# Autodesk Inventor assembly: A2017_T2_13
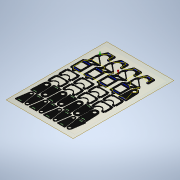
[picture p0: Inventor's stored thumbnail of the model, 180x180]
Saved by Autodesk Inventor 2020 (Build 240168000, 168)
## iProperties
Created: 2021-08-27
Part Number: A2017_T2_13
Document SubType Name: Assembly
Designer: Masato
Author: Masato
## Documents named in this file (6)
- D:\GitHub\inventor\SUSTAINA-OP\Cam\A2017_T2_13.iam
- D:\GitHub\inventor\SUSTAINA-OP\Cam\DisposableBoard.ipt
- D:\GitHub\inventor\SUSTAINA-OP\LowerBody\Foot\Foot_front_frame.ipt
- D:\GitHub\inventor\SUSTAINA-OP\LowerBody\Foot\Foot_back_frame.ipt
- D:\GitHub\inventor\SUSTAINA-OP\LowerBody\Ankle\Ankle_side_frame.ipt
- D:\GitHub\inventor\SUSTAINA-OP\LowerBody\Ankle\Ankle_back_frame.ipt
## Components (29 placed, 5 different names)
1. DisposableBoard:1 — メイト:2, メイト:1, フラッシュ:1, フラッシュ:2, メイト:4, メイト:5, メイト:6, メイト:7, 正接:1, メイト:9, メイト:10, メイト:11, メイト:12, メイト:13, メイト:15, メイト:16, メイト:18, メイト:21
2. Foot_back_frame:7 — メイト:18, メイト:19, メイト:20
3. Foot_back_frame:8 — メイト:21, メイト:22, メイト:23
4. Foot_front_frame:2 — メイト:7, メイト:8, 正接:1, 正接:3
5. Foot_front_frame:1 — メイト:4, メイト:5, メイト:6, メイト:8, 正接:2
6. Foot_front_frame:3
7. Foot_front_frame:4
8. Foot_front_frame:5
9. Foot_front_frame:6
10. Foot_front_frame:7 — メイト:19
11. Foot_front_frame:8
12. Foot_back_frame:1 — メイト:10, メイト:14, 正接:3
13. Foot_back_frame:2 — メイト:9, 正接:2, メイト:13, メイト:14, 正接:4
14. Foot_back_frame:3
15. Foot_back_frame:4
16. Foot_back_frame:5 — メイト:20
17. Foot_back_frame:6
18. Ankle_back_frame:1 — メイト:11, 正接:4, メイト:15
19. Ankle_back_frame:2 — メイト:17
20. Ankle_back_frame:3
21. Ankle_back_frame:4
22. Ankle_back_frame:5
23. Ankle_back_frame:6
24. Ankle_back_frame:7
25. Ankle_back_frame:8 — メイト:23
26. Ankle_side_frame:1 — メイト:12, メイト:16, メイト:17
27. Ankle_side_frame:2
28. Ankle_side_frame:3
29. Ankle_side_frame:4 — メイト:22
## Component patterns: (4 elements, first: Foot_front_frame:2 + Foot_front_frame:1), (3 elements, first: Foot_back_frame:1 + Foot_back_frame:2), (8 elements, first: Ankle_back_frame:1), (4 elements, first: Ankle_side_frame:1)
## Relationships (28: Mate 22, Tangent 4, Flush 2)
- メイト:2 [Mate]: DisposableBoard:1
- メイト:1 [Mate]: DisposableBoard:1
- フラッシュ:1 [Flush]: DisposableBoard:1
- フラッシュ:2 [Flush]: DisposableBoard:1
- メイト:4 [Mate]: DisposableBoard:1 ↔ Foot_front_frame:1
- メイト:5 [Mate] (2 mm): DisposableBoard:1 ↔ Foot_front_frame:1
- メイト:6 [Mate] (2 mm): DisposableBoard:1 ↔ Foot_front_frame:1
- メイト:7 [Mate]: DisposableBoard:1 ↔ Foot_front_frame:2
- メイト:8 [Mate] (2.5 mm): Foot_front_frame:2 ↔ Foot_front_frame:1
- 正接:1 [Tangent] (2 mm): DisposableBoard:1 ↔ Foot_front_frame:2
- メイト:9 [Mate]: DisposableBoard:1 ↔ Foot_back_frame:2
- メイト:10 [Mate]: DisposableBoard:1 ↔ Foot_back_frame:1
- メイト:11 [Mate]: DisposableBoard:1 ↔ Ankle_back_frame:1
- メイト:12 [Mate]: DisposableBoard:1 ↔ Ankle_side_frame:1
- 正接:2 [Tangent] (2.5 mm): Foot_front_frame:1 ↔ Foot_back_frame:2
- メイト:13 [Mate] (2 mm): DisposableBoard:1 ↔ Foot_back_frame:2
- メイト:14 [Mate] (2.5 mm): Foot_back_frame:1 ↔ Foot_back_frame:2
- 正接:3 [Tangent] (2.5 mm): Foot_front_frame:2 ↔ Foot_back_frame:1
- 正接:4 [Tangent] (2.5 mm): Foot_back_frame:2 ↔ Ankle_back_frame:1
- メイト:15 [Mate] (2 mm): DisposableBoard:1 ↔ Ankle_back_frame:1
- メイト:16 [Mate] (2 mm): DisposableBoard:1 ↔ Ankle_side_frame:1
- メイト:17 [Mate] (2.5 mm): Ankle_back_frame:2 ↔ Ankle_side_frame:1
- メイト:18 [Mate]: DisposableBoard:1 ↔ Foot_back_frame:7
- メイト:19 [Mate] (2.5 mm): Foot_back_frame:7 ↔ Foot_front_frame:7
- メイト:20 [Mate] (2.5 mm): Foot_back_frame:7 ↔ Foot_back_frame:5
- メイト:21 [Mate]: DisposableBoard:1 ↔ Foot_back_frame:8
- メイト:22 [Mate] (3 mm): Foot_back_frame:8 ↔ Ankle_side_frame:4
- メイト:23 [Mate] (3 mm): Foot_back_frame:8 ↔ Ankle_back_frame:8
